# Autodesk Inventor assembly: Plasma-flange-on-support
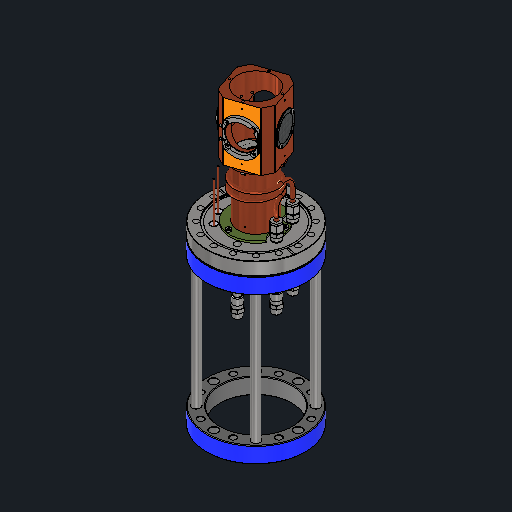
[picture p0: Inventor's stored thumbnail of the model, 512x512]
Saved by Autodesk Inventor 2025 (Build 290162000, 162)
## iProperties
Created: 2024-05-24
Part Number: Plasma-flange-on-support
Document SubType Name: Assembly
Designer: kuzmin
Author: kuzmin
## Documents named in this file (4)
- C:\Users\queezz\Dropbox\Drawings\PIHTI\Scaffolding\Plasma-flange-on-support.iam
- C:\Users\queezz\Dropbox\Drawings\PIHTI\Scaffolding\Plasma-flange-support.iam
- C:\Users\queezz\Dropbox\Drawings\PIHTI\Plasma Vessel\Plasma-Flange-2024\cathode-box-on-a-flange.iam
- C:\Users\queezz\Dropbox\Drawings\PIHTI\Plasma Vessel\Plasma-Box\Plasma-box-hayashi-aka-upgrade.iam
## Components (3 placed, 3 different names)
1. Plasma-flange-support:1 [sub-assembly] — Rotational:1, Mate:1
2. cathode-box-on-a-flange:1 [sub-assembly] — Rotational:1, Mate:1, Rotational:2
3. Plasma-box-hayashi-aka-upgrade:1 [sub-assembly] — Rotational:2
## Relationships (3: RevoluteJoint 2, Mate 1)
- Rotational:1 [RevoluteJoint]: Plasma-flange-support:1 ↔ cathode-box-on-a-flange:1
- Mate:1: Plasma-flange-support:1 ↔ cathode-box-on-a-flange:1
- Rotational:2 [RevoluteJoint]: cathode-box-on-a-flange:1 ↔ Plasma-box-hayashi-aka-upgrade:1
